# Autodesk Inventor assembly: Main Body
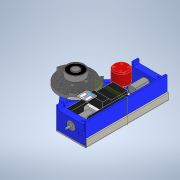
[picture p0: Inventor's stored thumbnail of the model, 180x180]
Saved by Autodesk Inventor 2022 (Build 260153000, 153)
## iProperties
Created: 2022-08-09
Part Number: Main Body
Document SubType Name: Assembly
Designer: Nick
Mass: 1318.27 g
Surface Area: 1845.37 cm^2
Volume: 451.196 cm^3
Density: 2.92172 g/cm^3
Author: Nick
## Documents named in this file (16)
- Y:\Projects\BattleBot\Main Body.iam
- Y:\Projects\BattleBot\Battery.ipt
- Y:\Projects\BattleBot\ESC.ipt
- Y:\Projects\BattleBot\Motor.ipt
- Y:\Projects\BattleBot\RC Reciever.ipt
- Y:\Projects\BattleBot\Base Plate.ipt
- Y:\Projects\BattleBot\Weapon.ipt
- Y:\Projects\BattleBot\Unmodified Motor.ipt
- Y:\Projects\BattleBot\Brushed ESC.ipt
- Y:\Projects\BattleBot\Motor Mount.ipt
- Y:\Projects\BattleBot\Wheel.ipt
- Y:\Projects\BattleBot\6201 Bearing.ipt
- Y:\Projects\BattleBot\Pulley.ipt
- Y:\Projects\BattleBot\6901 Bearing.ipt
- Y:\Projects\BattleBot\pulley flange.ipt
- Y:\Projects\BattleBot\GT2 Pulley 16T.ipt
## Components (20 placed, 15 different names)
1. Battery:1 — Mate:93, Mate:94, Mate:100, Mate:101
2. ESC:1 — Mate:84, Mate:85, Mate:91, Mate:101
3. RC Reciever:1 — Mate:94
4. Base Plate:1 — Flush:16, Mate:42, Mate:95, Insert:15
5. Weapon:1 — Mate:97, Mate:98
6. Unmodified Motor:1 — Mate:61, Insert:16
7. Motor:2 — Insert:8, Angle:1, Mate:100
8. Motor:3 — Insert:2, Insert:4, Angle:2
9. Brushed ESC:1 — Mate:83, Mate:89, Mate:90
10. Brushed ESC:2 — Mate:87, Mate:88
11. Motor Mount:2 — Insert:2, Flush:16, Mate:42, Insert:8, Mate:68, Mate:69, Flush:17, Angle:1, Angle:2, Mate:83, Mate:84, Mate:85, Mate:87, Mate:88, Mate:89, Mate:90, Mate:91, Mate:93, Mate:95, Mate:102
12. Base Plate:2 — Mate:61, Mate:68, Mate:69, Flush:17, Mate:99
13. Wheel:1
14. Wheel:2 — Insert:4
15. 6201 Bearing:2 — Mate:98, Mate:99
16. Pulley:1 — Insert:11, Insert:13, Insert:14, Mate:97
17. 6901 Bearing:1 — Insert:14, Insert:15
18. pulley flange:1 — Insert:11
19. pulley flange:2 — Insert:13
20. GT2 Pulley 16T:1 — Insert:16, Mate:102
## Relationships (33: Mate 21, Insert 8, Flush 2, Angle 2)
- Insert:2: Motor:3 ↔ Motor Mount:2
- Flush:16: Base Plate:1 ↔ Motor Mount:2
- Mate:42: Base Plate:1 ↔ Motor Mount:2
- Mate:61: Unmodified Motor:1 ↔ Base Plate:2
- Insert:4 (2 mm): Motor:3 ↔ Wheel:2
- Insert:8: Motor:2 ↔ Motor Mount:2
- Mate:68: Motor Mount:2 ↔ Base Plate:2
- Mate:69: Motor Mount:2 ↔ Base Plate:2
- Flush:17: Motor Mount:2 ↔ Base Plate:2
- Insert:11: Pulley:1 ↔ pulley flange:1
- Insert:13: Pulley:1 ↔ pulley flange:2
- Insert:14: Pulley:1 ↔ 6901 Bearing:1
- Angle:1 (0 deg): Motor:2 ↔ Motor Mount:2
- Angle:2 (0 deg): Motor:3 ↔ Motor Mount:2
- Mate:83: Brushed ESC:1 ↔ Motor Mount:2
- Mate:84: ESC:1 ↔ Motor Mount:2
- Mate:85: ESC:1 ↔ Motor Mount:2
- Mate:87: Brushed ESC:2 ↔ Motor Mount:2
- Mate:88 (5 mm): Brushed ESC:2 ↔ Motor Mount:2
- Mate:89 (5 mm): Brushed ESC:1 ↔ Motor Mount:2
- Mate:90: Brushed ESC:1 ↔ Motor Mount:2
- Mate:91 (5 mm): ESC:1 ↔ Motor Mount:2
- Mate:93: Battery:1 ↔ Motor Mount:2
- Mate:94: Battery:1 ↔ RC Reciever:1
- Mate:95: Base Plate:1 ↔ Motor Mount:2
- Insert:15: Base Plate:1 ↔ 6901 Bearing:1
- Insert:16: Unmodified Motor:1 ↔ GT2 Pulley 16T:1
- Mate:97: Weapon:1 ↔ Pulley:1
- Mate:98: Weapon:1 ↔ 6201 Bearing:2
- Mate:99: Base Plate:2 ↔ 6201 Bearing:2
- Mate:100 (5 mm): Battery:1 ↔ Motor:2
- Mate:101: Battery:1 ↔ ESC:1
- Mate:102: Motor Mount:2 ↔ GT2 Pulley 16T:1
